# Autodesk Inventor assembly: tester
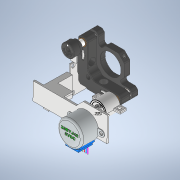
[picture p0: Inventor's stored thumbnail of the model, 180x180]
Saved by Autodesk Inventor 2020.2 (Build 242310000, 310)
## iProperties
Created: 2020-02-18
Part Number: tester
Document SubType Name: Assembly
Designer: ColinP
Author: ColinP
## Documents named in this file (5)
- C:\Users\ColinP\Documents\Inventor\steppermotoriqc\SteppermotorMirror\tester.iam
- C:\Users\ColinP\Documents\Inventor\steppermotoriqc\SteppermotorMirror\KM100-Step.ipt
- C:\Users\ColinP\Documents\Inventor\steppermotoriqc\SteppermotorMirror\socket.ipt
- C:\Users\ColinP\Documents\Inventor\steppermotoriqc\28BYJ-48 – 5V Stepper Motor\28BYJ-48 – 5V Stepper Motor.ipt
- C:\Users\ColinP\Documents\Inventor\steppermotoriqc\SteppermotorMirror\Shelf_half_left.ipt
## Components (5 placed, 4 different names)
1. KM100-Step:1 — Mate:1, Mate:2, Insert:1
2. Shelf_half_left:1 — Mate:1, Mate:2, Mate:4, Mate:5, Mate:6
3. 28BYJ-48 – 5V Stepper Motor:1 — Mate:4, Mate:5, Mate:6
4. socket:2 — Insert:1, Mate:7, Mate:8
5. socket:3 — Mate:7, Mate:8
## Relationships (8: Mate 7, Insert 1)
- Mate:1: KM100-Step:1 ↔ Shelf_half_left:1
- Mate:2: KM100-Step:1 ↔ Shelf_half_left:1
- Mate:4: Shelf_half_left:1 ↔ 28BYJ-48 – 5V Stepper Motor:1
- Insert:1: KM100-Step:1 ↔ socket:2
- Mate:5: Shelf_half_left:1 ↔ 28BYJ-48 – 5V Stepper Motor:1
- Mate:6: Shelf_half_left:1 ↔ 28BYJ-48 – 5V Stepper Motor:1
- Mate:7: socket:2 ↔ socket:3
- Mate:8: socket:2 ↔ socket:3
